# Autodesk Inventor assembly: ГЛАЗ НОВЫЙ СБОРКА_ЗЕРКАЛО_ЗЕРКАЛО
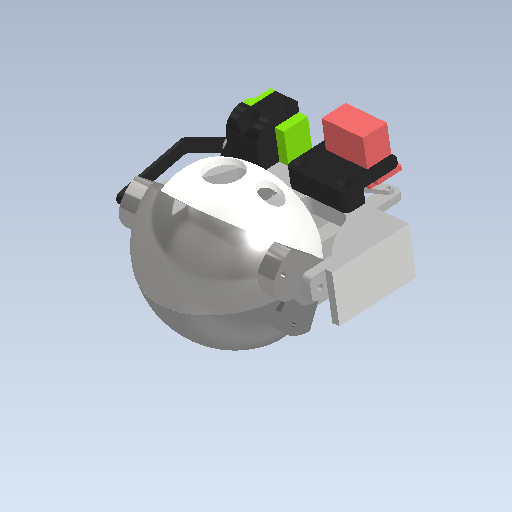
[picture p0: Inventor's stored thumbnail of the model, 512x512]
Saved by Autodesk Inventor 2020 (Build 240168000, 168)
## iProperties
Created: 2022-02-16
Part Number: ГЛАЗ НОВЫЙ СБОРКА_ЗЕРКАЛО_ЗЕРКАЛО
Document SubType Name: Assembly
Designer: HP
Author: Администратор
## Documents named in this file (14)
- C:\Users\HP\Downloads\ГЛАЗ НОВЫЙ СБОРКА_ЗЕРКАЛО_ЗЕРКАЛО.iam
- C:\Users\HP\Downloads\шатун движенияглаза_ЗЕРКАЛО_ЗЕРКАЛО.ipt
- C:\Users\HP\Downloads\связующий сервы движения глаз_ЗЕРКАЛО_ЗЕРКАЛО.ipt
- C:\Users\HP\Downloads\связующий сервы век_ЗЕРКАЛО_ЗЕРКАЛО.ipt
- C:\Users\HP\Downloads\нижнее веко_ЗЕРКАЛО_ЗЕРКАЛО.ipt
- C:\Users\HP\Downloads\держалка сервы движения глаз_ЗЕРКАЛО_ЗЕРКАЛО.ipt
- C:\Users\HP\Downloads\держалка сервы век_ЗЕРКАЛО_ЗЕРКАЛО.ipt
- C:\Users\HP\Downloads\держалка глаза_ЗЕРКАЛО_ЗЕРКАЛО.ipt
- C:\Users\HP\Downloads\верхнее веко_ЗЕРКАЛО_ЗЕРКАЛО.ipt
- C:\Users\HP\Downloads\SERVO_ЗЕРКАЛО_ЗЕРКАЛО.ipt
- C:\Users\HP\Downloads\нижний шатун век_ЗЕРКАЛО_ЗЕРКАЛО.ipt
- C:\Users\HP\Downloads\зрачок_ЗЕРКАЛО_ЗЕРКАЛО.ipt
- C:\Users\HP\Downloads\белок глаза_ЗЕРКАЛО_ЗЕРКАЛО_ЗЕРКАЛО.ipt
- C:\Users\HP\Downloads\верхний шатун века_ЗЕРКАЛО1_ЗЕРКАЛО_ЗЕРКАЛО.ipt
## Components (14 placed, 13 different names)
1. шатун движенияглаза_ЗЕРКАЛО_ЗЕРКАЛО:1 — Совмещение:30, Совмещение:31, Совмещение:46, Совмещение:47
2. связующий сервы движения глаз_ЗЕРКАЛО_ЗЕРКАЛО:1 — Совмещение:20, Совмещение:43, Совмещение:16, Совмещение:44
3. связующий сервы век_ЗЕРКАЛО_ЗЕРКАЛО:1 — Совмещение:30, Совмещение:31, Совмещение:38
4. нижнее веко_ЗЕРКАЛО_ЗЕРКАЛО:1 — Совмещение:5, Совмещение:6, Совмещение:7, Совмещение:8, Совмещение:9, Совмещение:41, Совмещение:42
5. держалка сервы движения глаз_ЗЕРКАЛО_ЗЕРКАЛО:1 — Совмещение:32, Совмещение:33, Совмещение:34, Совмещение:35, Совмещение:36, Совмещение:37
6. держалка сервы век_ЗЕРКАЛО_ЗЕРКАЛО:1 — Совмещение:21, Совмещение:22, Совмещение:23
7. держалка глаза_ЗЕРКАЛО_ЗЕРКАЛО:1 — Совмещение:5, Совмещение:6, Совмещение:7, Совмещение:32, Совмещение:33, Совмещение:34, Совмещение:10, Совмещение:18, Совмещение:19, Совмещение:45, Совмещение:48, Угол:1
8. верхнее веко_ЗЕРКАЛО_ЗЕРКАЛО:1 — Совмещение:8, Совмещение:9, Совмещение:10, Совмещение:13, Совмещение:14
9. SERVO_ЗЕРКАЛО_ЗЕРКАЛО:1 — Совмещение:18, Совмещение:19, Совмещение:20, Совмещение:21, Совмещение:22, Совмещение:23, Совмещение:43, Угол:1
10. SERVO_ЗЕРКАЛО_ЗЕРКАЛО:2 — Совмещение:35, Совмещение:36, Совмещение:37, Совмещение:38
11. нижний шатун век_ЗЕРКАЛО_ЗЕРКАЛО:1 — Совмещение:13, Совмещение:14, Совмещение:16
12. зрачок_ЗЕРКАЛО_ЗЕРКАЛО:1 — Совмещение:39, Совмещение:40
13. белок глаза_ЗЕРКАЛО_ЗЕРКАЛО_ЗЕРКАЛО:1 — Совмещение:39, Совмещение:40, Совмещение:45, Совмещение:46, Совмещение:47, Совмещение:48
14. верхний шатун века_ЗЕРКАЛО1_ЗЕРКАЛО_ЗЕРКАЛО:1 — Совмещение:41, Совмещение:42, Совмещение:44
## Relationships (35: Mate 34, Angle 1)
- Совмещение:30 [Mate]: шатун движенияглаза_ЗЕРКАЛО_ЗЕРКАЛО:1 ↔ связующий сервы век_ЗЕРКАЛО_ЗЕРКАЛО:1
- Совмещение:31 [Mate]: шатун движенияглаза_ЗЕРКАЛО_ЗЕРКАЛО:1 ↔ связующий сервы век_ЗЕРКАЛО_ЗЕРКАЛО:1
- Совмещение:5 [Mate]: нижнее веко_ЗЕРКАЛО_ЗЕРКАЛО:1 ↔ держалка глаза_ЗЕРКАЛО_ЗЕРКАЛО:1
- Совмещение:6 [Mate]: нижнее веко_ЗЕРКАЛО_ЗЕРКАЛО:1 ↔ держалка глаза_ЗЕРКАЛО_ЗЕРКАЛО:1
- Совмещение:7 [Mate]: нижнее веко_ЗЕРКАЛО_ЗЕРКАЛО:1 ↔ держалка глаза_ЗЕРКАЛО_ЗЕРКАЛО:1
- Совмещение:32 [Mate]: держалка сервы движения глаз_ЗЕРКАЛО_ЗЕРКАЛО:1 ↔ держалка глаза_ЗЕРКАЛО_ЗЕРКАЛО:1
- Совмещение:33 [Mate]: держалка сервы движения глаз_ЗЕРКАЛО_ЗЕРКАЛО:1 ↔ держалка глаза_ЗЕРКАЛО_ЗЕРКАЛО:1
- Совмещение:34 [Mate]: держалка сервы движения глаз_ЗЕРКАЛО_ЗЕРКАЛО:1 ↔ держалка глаза_ЗЕРКАЛО_ЗЕРКАЛО:1
- Совмещение:8 [Mate]: нижнее веко_ЗЕРКАЛО_ЗЕРКАЛО:1 ↔ верхнее веко_ЗЕРКАЛО_ЗЕРКАЛО:1
- Совмещение:9 [Mate]: нижнее веко_ЗЕРКАЛО_ЗЕРКАЛО:1 ↔ верхнее веко_ЗЕРКАЛО_ЗЕРКАЛО:1
- Совмещение:10 [Mate]: держалка глаза_ЗЕРКАЛО_ЗЕРКАЛО:1 ↔ верхнее веко_ЗЕРКАЛО_ЗЕРКАЛО:1
- Совмещение:18 [Mate]: держалка глаза_ЗЕРКАЛО_ЗЕРКАЛО:1 ↔ SERVO_ЗЕРКАЛО_ЗЕРКАЛО:1
- Совмещение:19 [Mate]: держалка глаза_ЗЕРКАЛО_ЗЕРКАЛО:1 ↔ SERVO_ЗЕРКАЛО_ЗЕРКАЛО:1
- Совмещение:20 [Mate]: связующий сервы движения глаз_ЗЕРКАЛО_ЗЕРКАЛО:1 ↔ SERVO_ЗЕРКАЛО_ЗЕРКАЛО:1
- Совмещение:21 [Mate]: держалка сервы век_ЗЕРКАЛО_ЗЕРКАЛО:1 ↔ SERVO_ЗЕРКАЛО_ЗЕРКАЛО:1
- Совмещение:22 [Mate]: держалка сервы век_ЗЕРКАЛО_ЗЕРКАЛО:1 ↔ SERVO_ЗЕРКАЛО_ЗЕРКАЛО:1
- Совмещение:23 [Mate]: держалка сервы век_ЗЕРКАЛО_ЗЕРКАЛО:1 ↔ SERVO_ЗЕРКАЛО_ЗЕРКАЛО:1
- Совмещение:43 [Mate]: связующий сервы движения глаз_ЗЕРКАЛО_ЗЕРКАЛО:1 ↔ SERVO_ЗЕРКАЛО_ЗЕРКАЛО:1
- Совмещение:35 [Mate]: держалка сервы движения глаз_ЗЕРКАЛО_ЗЕРКАЛО:1 ↔ SERVO_ЗЕРКАЛО_ЗЕРКАЛО:2
- Совмещение:36 [Mate]: держалка сервы движения глаз_ЗЕРКАЛО_ЗЕРКАЛО:1 ↔ SERVO_ЗЕРКАЛО_ЗЕРКАЛО:2
- Совмещение:37 [Mate]: держалка сервы движения глаз_ЗЕРКАЛО_ЗЕРКАЛО:1 ↔ SERVO_ЗЕРКАЛО_ЗЕРКАЛО:2
- Совмещение:38 [Mate]: связующий сервы век_ЗЕРКАЛО_ЗЕРКАЛО:1 ↔ SERVO_ЗЕРКАЛО_ЗЕРКАЛО:2
- Совмещение:13 [Mate]: верхнее веко_ЗЕРКАЛО_ЗЕРКАЛО:1 ↔ нижний шатун век_ЗЕРКАЛО_ЗЕРКАЛО:1
- Совмещение:14 [Mate]: верхнее веко_ЗЕРКАЛО_ЗЕРКАЛО:1 ↔ нижний шатун век_ЗЕРКАЛО_ЗЕРКАЛО:1
- Совмещение:16 [Mate]: связующий сервы движения глаз_ЗЕРКАЛО_ЗЕРКАЛО:1 ↔ нижний шатун век_ЗЕРКАЛО_ЗЕРКАЛО:1
- Совмещение:39 [Mate]: зрачок_ЗЕРКАЛО_ЗЕРКАЛО:1 ↔ белок глаза_ЗЕРКАЛО_ЗЕРКАЛО_ЗЕРКАЛО:1
- Совмещение:40 [Mate]: зрачок_ЗЕРКАЛО_ЗЕРКАЛО:1 ↔ белок глаза_ЗЕРКАЛО_ЗЕРКАЛО_ЗЕРКАЛО:1
- Совмещение:45 [Mate]: держалка глаза_ЗЕРКАЛО_ЗЕРКАЛО:1 ↔ белок глаза_ЗЕРКАЛО_ЗЕРКАЛО_ЗЕРКАЛО:1
- Совмещение:46 [Mate]: шатун движенияглаза_ЗЕРКАЛО_ЗЕРКАЛО:1 ↔ белок глаза_ЗЕРКАЛО_ЗЕРКАЛО_ЗЕРКАЛО:1
- Совмещение:47 [Mate]: шатун движенияглаза_ЗЕРКАЛО_ЗЕРКАЛО:1 ↔ белок глаза_ЗЕРКАЛО_ЗЕРКАЛО_ЗЕРКАЛО:1
- Совмещение:48 [Mate]: держалка глаза_ЗЕРКАЛО_ЗЕРКАЛО:1 ↔ белок глаза_ЗЕРКАЛО_ЗЕРКАЛО_ЗЕРКАЛО:1
- Совмещение:41 [Mate]: нижнее веко_ЗЕРКАЛО_ЗЕРКАЛО:1 ↔ верхний шатун века_ЗЕРКАЛО1_ЗЕРКАЛО_ЗЕРКАЛО:1
- Совмещение:42 [Mate]: нижнее веко_ЗЕРКАЛО_ЗЕРКАЛО:1 ↔ верхний шатун века_ЗЕРКАЛО1_ЗЕРКАЛО_ЗЕРКАЛО:1
- Совмещение:44 [Mate]: связующий сервы движения глаз_ЗЕРКАЛО_ЗЕРКАЛО:1 ↔ верхний шатун века_ЗЕРКАЛО1_ЗЕРКАЛО_ЗЕРКАЛО:1
- Угол:1 [Angle] (0 deg): держалка глаза_ЗЕРКАЛО_ЗЕРКАЛО:1 ↔ SERVO_ЗЕРКАЛО_ЗЕРКАЛО:1
